# Autodesk Inventor assembly: Ensamble_completo
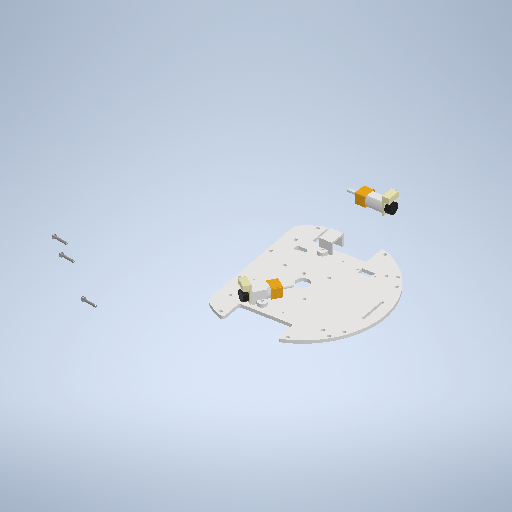
[picture p0: Inventor's stored thumbnail of the model, 512x512]
Saved by Autodesk Inventor 2025.3 (Build 293356030, 356C)
## iProperties
Created: 2025-10-21
Part Number: Ensamble_completo
Document SubType Name: Assembly
Designer: brene
Author: brene
## Documents named in this file (6)
- D:\OneDrive - Estudiantes ITCR\Documentos\GitHub\Atta-Bot-STEM\Chasis\Rediseño_Diego&Carlos\Carcasa 4.0 Rediseño\Ensamble_completo.iam
- D:\OneDrive - Estudiantes ITCR\Documentos\GitHub\Atta-Bot-STEM\Chasis\Rediseño_Diego&Carlos\Carcasa 4.0 Rediseño\base_chasis_v6\base_chasis_v4-dimsAjustadas.ipt
- D:\OneDrive - Estudiantes ITCR\Documentos\GitHub\Atta-Bot-STEM\Chasis\Rediseño_Diego&Carlos\Carcasa 4.0 Rediseño\base_chasis_v6.ipt
- D:\OneDrive - Estudiantes ITCR\Documentos\GitHub\Atta-Bot-STEM\Chasis\Rediseño_Diego&Carlos\motor.ipt
- D:\OneDrive - Estudiantes ITCR\Documentos\GitHub\Atta-Bot-STEM\Chasis\Rediseño_Diego&Carlos\soporteMotor_MIR.ipt
- D:\OneDrive - Estudiantes ITCR\Documentos\GitHub\Atta-Bot-STEM\Chasis\Rediseño_Diego&Carlos\Content Center Files\en-US\ISO 4762(2)\ISO 4762 - M2 x 12ISO.ipt
## Components (9 placed, 4 different names)
1. base_chasis_v4-dimsAjustadas:1 — Mate:1, Mate:2, Mate:3, Mate:4, Mate:5, Mate:7, Mate:9
2. soporteMotor_MIR:1 — Mate:1, Mate:2, Mate:8
3. soporteMotor_MIR:2 — Mate:3, Mate:4, Mate:6, Tangent:1, Mate:9, Mate:10, Mate:11
4. motor:1 — Mate:7, Mate:8
5. motor:2 — Mate:5, Mate:6, Tangent:1
6. ISO 4762 M2 x 12:1 — Mate:10, Mate:11
7. ISO 4762 M2 x 12:2
8. ISO 4762 M2 x 12:3
9. ISO 4762 M2 x 12:4
## Relationships (12: Mate 11, Tangent 1)
- Mate:1: base_chasis_v4-dimsAjustadas:1 ↔ soporteMotor_MIR:1
- Mate:2: base_chasis_v4-dimsAjustadas:1 ↔ soporteMotor_MIR:1
- Mate:3: base_chasis_v4-dimsAjustadas:1 ↔ soporteMotor_MIR:2
- Mate:4: base_chasis_v4-dimsAjustadas:1 ↔ soporteMotor_MIR:2
- Mate:5: base_chasis_v4-dimsAjustadas:1 ↔ motor:2
- Mate:6: soporteMotor_MIR:2 ↔ motor:2
- Tangent:1: soporteMotor_MIR:2 ↔ motor:2
- Mate:7: base_chasis_v4-dimsAjustadas:1 ↔ motor:1
- Mate:8: soporteMotor_MIR:1 ↔ motor:1
- Mate:9: base_chasis_v4-dimsAjustadas:1 ↔ soporteMotor_MIR:2
- Mate:10: soporteMotor_MIR:2 ↔ ISO 4762 M2 x 12:1
- Mate:11: soporteMotor_MIR:2 ↔ ISO 4762 M2 x 12:1
